# Autodesk Inventor assembly: SPE2V1 Baranda
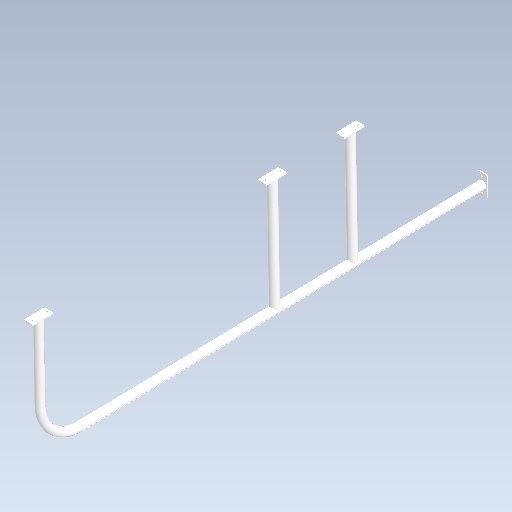
[picture p0: Inventor's stored thumbnail of the model, 512x512]
Saved by Autodesk Inventor 2021.2 (Build 252289000, 289)
## iProperties
Created: 2026-06-02
Part Number: SPE2V1 Baranda
Document SubType Name: Assembly
Designer: nelso
Author: nelso
## Documents named in this file (4)
- C:\Users\nelso\Documents\Escritorio\Soporte-Paciente-Espinografia\Workspace\SPE2V1 Baranda.iam
- C:\Users\nelso\Documents\Escritorio\Soporte-Paciente-Espinografia\Workspace\SP13V1 Tubo Baranda.ipt
- C:\Users\nelso\Documents\Escritorio\Soporte-Paciente-Espinografia\Workspace\SP12V1 Agarre Baranda.ipt
- C:\Users\nelso\Documents\Escritorio\Soporte-Paciente-Espinografia\Workspace\SP11V1 Planchuela Baranda.ipt
## Components (7 placed, 3 different names)
1. SP13V1 Tubo Baranda:1 — Mate:3, Mate:4, Mate:5, Coincidencia:15, Coincidencia:16, Coincidencia:17, Coincidencia:18, Mate:20, Mate:21
2. SP12V1 Agarre Baranda:1 — Mate:4, Mate:7, Mate:9, Mate:10, Mate:20
3. SP12V1 Agarre Baranda:2 — Mate:3, Mate:6, Mate:12, Mate:13, Mate:21
4. SP11V1 Planchuela Baranda:1 — Mate:8, Mate:9, Mate:10
5. SP11V1 Planchuela Baranda:2 — Coincidencia:14, Coincidencia:15, Coincidencia:16
6. SP11V1 Planchuela Baranda:3 — Mate:11, Mate:12, Mate:13
7. SP11V1 Planchuela Baranda:4 — Coincidencia:17, Coincidencia:18, Coincidencia:19
## Relationships (19: Mate 19)
- Mate:3 (-500 mm): SP13V1 Tubo Baranda:1 ↔ SP12V1 Agarre Baranda:2
- Mate:4 (-800 mm): SP13V1 Tubo Baranda:1 ↔ SP12V1 Agarre Baranda:1
- Mate:5: SP13V1 Tubo Baranda:1
- Mate:6: SP12V1 Agarre Baranda:2
- Mate:7: SP12V1 Agarre Baranda:1
- Mate:8: SP11V1 Planchuela Baranda:1
- Mate:9: SP12V1 Agarre Baranda:1 ↔ SP11V1 Planchuela Baranda:1
- Mate:10: SP12V1 Agarre Baranda:1 ↔ SP11V1 Planchuela Baranda:1
- Mate:11: SP11V1 Planchuela Baranda:3
- Mate:12: SP12V1 Agarre Baranda:2 ↔ SP11V1 Planchuela Baranda:3
- Mate:13: SP12V1 Agarre Baranda:2 ↔ SP11V1 Planchuela Baranda:3
- Coincidencia:14 [Mate]: SP11V1 Planchuela Baranda:2
- Coincidencia:15 [Mate]: SP13V1 Tubo Baranda:1 ↔ SP11V1 Planchuela Baranda:2
- Coincidencia:16 [Mate]: SP13V1 Tubo Baranda:1 ↔ SP11V1 Planchuela Baranda:2
- Coincidencia:17 [Mate]: SP13V1 Tubo Baranda:1 ↔ SP11V1 Planchuela Baranda:4
- Coincidencia:18 [Mate]: SP13V1 Tubo Baranda:1 ↔ SP11V1 Planchuela Baranda:4
- Coincidencia:19 [Mate]: SP11V1 Planchuela Baranda:4
- Mate:20: SP13V1 Tubo Baranda:1 ↔ SP12V1 Agarre Baranda:1
- Mate:21: SP13V1 Tubo Baranda:1 ↔ SP12V1 Agarre Baranda:2
